# Autodesk Inventor assembly: v.3
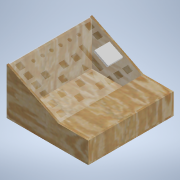
[picture p0: Inventor's stored thumbnail of the model, 180x180]
Saved by Autodesk Inventor 2021.1 (Build 251245000, 245)
## iProperties
Created: 2020-08-02
Part Number: v.3
Document SubType Name: Assembly
Designer: adick
Author: adick
## Documents named in this file (8)
- C:\Users\adick\Documents\Kerbal Kontroller\Inventor CAD\v.3.iam
- C:\Users\adick\Documents\Kerbal Kontroller\Inventor CAD\Parts\Sides.ipt
- C:\Users\adick\Documents\Kerbal Kontroller\Inventor CAD\Parts\Bottom.ipt
- C:\Users\adick\Documents\Kerbal Kontroller\Inventor CAD\Parts\Front.ipt
- C:\Users\adick\Documents\Kerbal Kontroller\Inventor CAD\Parts\Back.ipt
- C:\Users\adick\Documents\Kerbal Kontroller\Inventor CAD\Parts\Front Plywood.ipt
- C:\Users\adick\Documents\Kerbal Kontroller\Inventor CAD\Parts\Arm Rest.ipt
- C:\Users\adick\Documents\Kerbal Kontroller\Inventor CAD\Parts\Stage Keycap.ipt
## Components (8 placed, 7 different names)
1. Sides:1 — Mate:3, Mate:5
2. Bottom:1 — Mate:2
3. Front:1 — Mate:1
4. Back:1
5. Sides:2 — Mate:1, Mate:2, Mate:4
6. Front Plywood:1 — Mate:3, Mate:4, Mate:5, Mate:6, Mate:7
7. Arm Rest:1
8. Stage Keycap:1 — Mate:6, Mate:7
## Relationships (7: Mate 7)
- Mate:1: Front:1 ↔ Sides:2
- Mate:2: Bottom:1 ↔ Sides:2
- Mate:3: Sides:1 ↔ Front Plywood:1
- Mate:4: Sides:2 ↔ Front Plywood:1
- Mate:5: Sides:1 ↔ Front Plywood:1
- Mate:6: Front Plywood:1 ↔ Stage Keycap:1
- Mate:7: Front Plywood:1 ↔ Stage Keycap:1
